# Autodesk Inventor assembly: stilladssøjle
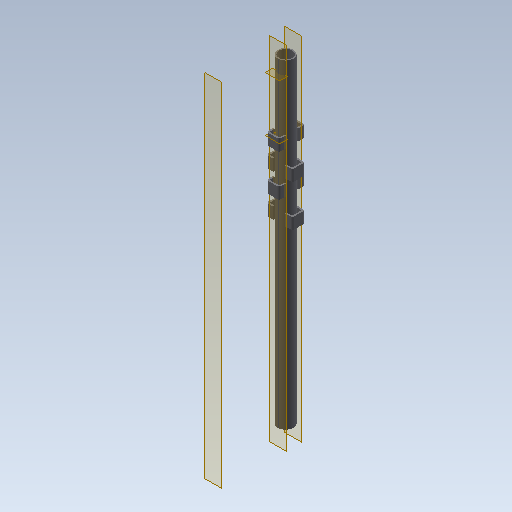
[picture p0: Inventor's stored thumbnail of the model, 512x512]
Saved by Autodesk Inventor 2020.1 (Build 241239000, 239)
## iProperties
Created: 2019-09-25
Part Number: stilladssøjle
Document SubType Name: Assembly
Designer: loppen
Mass: 4907.59 g
Surface Area: 3297.75 cm^2
Volume: 625.171 cm^3
Density: 7.85 g/cm^3
Author: loppen
## Documents named in this file (3)
- Y:\trappe\søjle\stilladssøjle.iam
- Y:\trappe\søjle\rør.ipt
- Y:\trappe\søjle\øre.ipt
## Components (9 placed, 2 different names)
1. rør:1 — Mate:1, Tangent:1, Mate:2, Tangent:2, Flush:2, Flush:5, Flush:7, Flush:8, Tangent:3, Tangent:4, Flush:11, Flush:12, Tangent:5, Tangent:6, Tangent:7, Mate:3, Mate:4, Tangent:8
2. øre:1 — Mate:1, Tangent:1, Flush:1, Flush:2, Flush:3, Flush:9, Flush:17
3. øre:2 — Mate:2, Tangent:2, Flush:1, Flush:10
4. øre:3 — Flush:7, Tangent:3, Flush:9
5. øre:4 — Flush:8, Tangent:4, Flush:10
6. øre:5 — Flush:11, Tangent:6, Flush:13, Flush:16, Flush:17
7. øre:6 — Flush:12, Tangent:5, Flush:13, Flush:15
8. øre:7 — Tangent:7, Mate:3, Flush:16
9. øre:8 — Tangent:8, Mate:4, Flush:15
## Relationships (29: Flush 17, Tangent 8, Mate 4)
- Mate:1: rør:1 ↔ øre:1
- Tangent:1: rør:1 ↔ øre:1
- Mate:2: rør:1 ↔ øre:2
- Tangent:2: rør:1 ↔ øre:2
- Flush:1 (-130 mm): øre:1 ↔ øre:2
- Flush:2 (-200 mm): rør:1 ↔ øre:1
- Flush:3 (160 mm): øre:1
- Flush:4 (-170.6 mm)
- Flush:5 (250 mm): rør:1
- [Flush] (-130 mm): øre:3 ↔ øre:4
- Flush:7: rør:1 ↔ øre:3
- Flush:8: rør:1 ↔ øre:4
- Tangent:3: rør:1 ↔ øre:3
- Tangent:4: rør:1 ↔ øre:4
- Flush:9: øre:1 ↔ øre:3
- Flush:10: øre:2 ↔ øre:4
- Flush:11: rør:1 ↔ øre:5
- Flush:12: rør:1 ↔ øre:6
- Tangent:5: rør:1 ↔ øre:6
- Tangent:6: rør:1 ↔ øre:5
- Flush:13 (-130 mm): øre:5 ↔ øre:6
- [Flush] (-130 mm): øre:7 ↔ øre:8
- Tangent:8: rør:1 ↔ øre:8
- Tangent:7: rør:1 ↔ øre:7
- Mate:3: rør:1 ↔ øre:7
- Mate:4: rør:1 ↔ øre:8
- Flush:15: øre:6 ↔ øre:8
- Flush:16: øre:5 ↔ øre:7
- Flush:17 (-82 mm): øre:1 ↔ øre:5
